# Autodesk Inventor assembly: HS 48T Gear, Circle_MIR
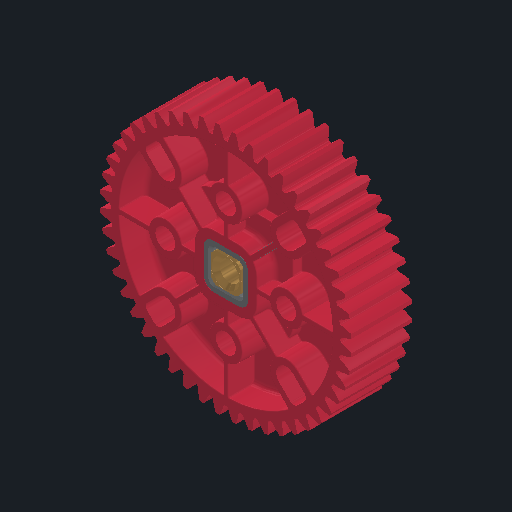
[picture p0: Inventor's stored thumbnail of the model, 512x512]
Saved by Autodesk Inventor 2026.2 (Build 302298000, 298)
## iProperties
Created: 2022-08-02
Part Number: HS 48T Gear, Circle_MIR
Document SubType Name: Assembly
Designer: sakin_wbdzdu1
Author: ylu12
## Documents named in this file (3)
- C:\Personal\Deprecated\VEX V5 Push Back\S-bot-two\CAD\VEX-CAD-Inventor-1.4.2\Motion\Gears\HS Gear\HS 48T Gear, Circle_MIR.iam
- C:\Personal\Deprecated\VEX V5 Push Back\S-bot-two\CAD\VEX-CAD-Inventor-1.4.2\Motion\HS Shaft Adapter Circle_MIR.ipt
- C:\Personal\Deprecated\VEX V5 Push Back\S-bot-two\CAD\VEX-CAD-Inventor-1.4.2\Motion\Gears\Reference Files\HS 48T Gear, No Insert_MIR.ipt
## Components (2 placed, 2 different names)
1. HS Shaft Adapter Circle_MIR:1 — Flush:1, Mate:2, Mate:1
2. HS 48T Gear, No Insert_MIR:1 — Mate:12, Mate:11, Flush:6
## Relationships (6: Mate 4, Flush 2)
- Flush:1 (-6.35 mm): HS Shaft Adapter Circle_MIR:1
- Mate:2: HS Shaft Adapter Circle_MIR:1
- Mate:1: HS Shaft Adapter Circle_MIR:1
- Mate:12: HS 48T Gear, No Insert_MIR:1
- Mate:11: HS 48T Gear, No Insert_MIR:1
- Flush:6: HS 48T Gear, No Insert_MIR:1
